# Autodesk Inventor assembly: 武器把手
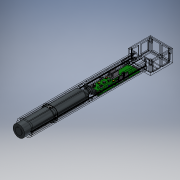
[picture p0: Inventor's stored thumbnail of the model, 180x180]
Saved by Autodesk Inventor 2017 (Build 210142000, 142)
## iProperties
Part Number: 武器把手
Material: 一般
Document SubType Name: Assembly
Designer: G
Author: G
## Documents named in this file (9)
- Z:\資料\公司資料\一江資訊\武器把手\武器把手.iam
- Z:\資料\公司資料\一江資訊\武器把手\手把A.ipt
- Z:\資料\公司資料\一江資訊\武器把手\28650凸.ipt
- Z:\資料\公司資料\一江資訊\武器把手\磁鐵A.ipt
- Z:\資料\公司資料\一江資訊\武器把手\C-FBPJ5-20P\C-FBPJ5-20P.iam
- Z:\資料\公司資料\一江資訊\武器把手\限位塊.ipt
- Z:\資料\公司資料\一江資訊\武器把手\box.ipt
- Z:\資料\公司資料\一江資訊\武器把手\電路板\電路板1.iam
- Z:\資料\公司資料\一江資訊\武器把手\磁鐵b.ipt
## Components (12 placed, 8 different names)
1. box:2 — 貼合:5, 貼合:6, 角度:3, 貼合:8, 貼合:9, 貼合:10
2. 28650凸:1 — 貼合:2, 貼合:3, 插入:3, 貼合:8
3. 磁鐵A:1 — 貼合:4, 角度:2, 貼合:7, 貼合:9
4. 28650凸:2 — 插入:4
5. 手把A:2
6. 限位塊:1 — 插入:2, 插入:3, 插入:4, 插入:5, 插入:6, 插入:7
7. C-FBPJ5-20P:1 [sub-assembly] — 插入:2
8. 磁鐵b:1 — 貼合:2, 貼合:3, 貼合:4, 角度:2, 角度:3, 貼合:7
9. 電路板1:1 [sub-assembly] — 貼合:5, 貼合:6, 貼合:10
10. C-FBPJ5-20P:2 [sub-assembly] — 插入:5
11. C-FBPJ5-20P:3 [sub-assembly] — 插入:6
12. C-FBPJ5-20P:4 [sub-assembly] — 插入:7
## Relationships (17: Mate 9, Insert 6, Angle 2)
- 插入:2 [Insert]: 限位塊:1 ↔ C-FBPJ5-20P:1
- 貼合:2 [Mate]: 28650凸:1 ↔ 磁鐵b:1
- 貼合:3 [Mate] (5 mm): 28650凸:1 ↔ 磁鐵b:1
- 貼合:4 [Mate]: 磁鐵A:1 ↔ 磁鐵b:1
- 角度:2 [Angle] (0 deg): 磁鐵A:1 ↔ 磁鐵b:1
- 貼合:5 [Mate]: box:2 ↔ 電路板1:1
- 貼合:6 [Mate]: box:2 ↔ 電路板1:1
- 插入:3 [Insert]: 28650凸:1 ↔ 限位塊:1
- 插入:4 [Insert]: 28650凸:2 ↔ 限位塊:1
- 角度:3 [Angle] (0 deg): box:2 ↔ 磁鐵b:1
- 貼合:7 [Mate]: 磁鐵A:1 ↔ 磁鐵b:1
- 貼合:8 [Mate]: box:2 ↔ 28650凸:1
- 貼合:9 [Mate] (3 mm): box:2 ↔ 磁鐵A:1
- 插入:5 [Insert]: 限位塊:1 ↔ C-FBPJ5-20P:2
- 插入:6 [Insert]: 限位塊:1 ↔ C-FBPJ5-20P:3
- 插入:7 [Insert]: 限位塊:1 ↔ C-FBPJ5-20P:4
- 貼合:10 [Mate]: box:2 ↔ 電路板1:1
